# Autodesk Inventor assembly: Ensamblaje1
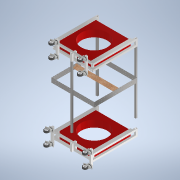
[picture p0: Inventor's stored thumbnail of the model, 180x180]
Saved by Autodesk Inventor 2020 (Build 240168000, 168)
## iProperties
Created: 2022-03-23
Part Number: Ensamblaje1
Document SubType Name: Assembly
Designer: aarco
Author: aarco
## Documents named in this file (8)
- C:\Users\aarco\Desktop\IDOM\Ensamblaje1.iam
- C:\Users\aarco\Desktop\IDOM\Latch.ipt
- C:\Users\aarco\Desktop\IDOM\SoporteBobina.ipt
- C:\Users\aarco\Desktop\IDOM\Madera.ipt
- C:\Users\aarco\Desktop\IDOM\Bobina.ipt
- C:\Users\aarco\Desktop\IDOM\Grid.ipt
- C:\Users\aarco\Desktop\IDOM\SoporteBobina_izq.ipt
- C:\Users\aarco\Desktop\IDOM\BPAB 1001 6150.ipt
## Components (18 placed, 7 different names)
1. Latch:1 — Rígido:1
2. SoporteBobina:1 — Coincidencia:1, Coincidencia:3, Coincidencia:4, Nivelación:1, Coincidencia:5, Coincidencia:7, Coincidencia:18, Nivelación:9, Nivelación:10, Coincidencia:24, Nivelación:13, Nivelación:14
3. Madera:1 — Rígido:1, Rígido:2, Coincidencia:13, Ángulo:1, Rígido:3, Rígido:4, Coincidencia:14, Coincidencia:15, Nivelación:8
4. Latch:2 — Rígido:2
5. Bobina:1 — Coincidencia:1, Coincidencia:3, Coincidencia:4
6. Grid:1 — Coincidencia:14, Coincidencia:15, Nivelación:8, Coincidencia:17, Coincidencia:18, Coincidencia:25
7. Bobina:2 — Coincidencia:20, Coincidencia:21, Coincidencia:22
8. Latch:3 — Rígido:3
9. Latch:4 — Rígido:4
10. SoporteBobina_izq:1 — Nivelación:9, Nivelación:10, Coincidencia:20, Coincidencia:21, Coincidencia:22, Coincidencia:23, Nivelación:11, Nivelación:12, Coincidencia:25
11. BPAB 1001 6150:1 — Coincidencia:23, Nivelación:11, Nivelación:12
12. BPAB 1001 6150:2
13. BPAB 1001 6150:3
14. BPAB 1001 6150:4
15. BPAB 1001 6150:6 — Coincidencia:24, Nivelación:13, Nivelación:14
16. BPAB 1001 6150:7
17. BPAB 1001 6150:8
18. BPAB 1001 6150:9
## Component patterns: (4 elements, first: BPAB 1001 6150:1), (4 elements, first: BPAB 1001 6150:6)
## Relationships (29: Mate 16, Flush 8, WeldJoint 4, Angle 1)
- Rígido:1 [WeldJoint]: Latch:1 ↔ Madera:1
- Rígido:2 [WeldJoint]: Madera:1 ↔ Latch:2
- Coincidencia:1 [Mate]: SoporteBobina:1 ↔ Bobina:1
- Coincidencia:3 [Mate]: SoporteBobina:1 ↔ Bobina:1
- Coincidencia:4 [Mate]: SoporteBobina:1 ↔ Bobina:1
- Nivelación:1 [Flush] (500 mm): SoporteBobina:1
- Coincidencia:5 [Mate]: SoporteBobina:1
- Coincidencia:7 [Mate]: SoporteBobina:1
- Coincidencia:13 [Mate]: Madera:1
- Ángulo:1 [Angle] (0 deg): Madera:1
- Rígido:3 [WeldJoint]: Madera:1 ↔ Latch:3
- Rígido:4 [WeldJoint]: Madera:1 ↔ Latch:4
- Coincidencia:14 [Mate]: Madera:1 ↔ Grid:1
- Coincidencia:15 [Mate] (400 mm): Madera:1 ↔ Grid:1
- Nivelación:8 [Flush]: Madera:1 ↔ Grid:1
- Coincidencia:17 [Mate]: Grid:1
- Coincidencia:18 [Mate] (800 mm): SoporteBobina:1 ↔ Grid:1
- Nivelación:9 [Flush]: SoporteBobina:1 ↔ SoporteBobina_izq:1
- Nivelación:10 [Flush]: SoporteBobina:1 ↔ SoporteBobina_izq:1
- Coincidencia:20 [Mate]: Bobina:2 ↔ SoporteBobina_izq:1
- Coincidencia:21 [Mate]: Bobina:2 ↔ SoporteBobina_izq:1
- Coincidencia:22 [Mate]: Bobina:2 ↔ SoporteBobina_izq:1
- Coincidencia:23 [Mate]: SoporteBobina_izq:1 ↔ BPAB 1001 6150:1
- Nivelación:11 [Flush] (-2.5 mm): SoporteBobina_izq:1 ↔ BPAB 1001 6150:1
- Nivelación:12 [Flush] (2.5 mm): SoporteBobina_izq:1 ↔ BPAB 1001 6150:1
- Coincidencia:24 [Mate]: SoporteBobina:1 ↔ BPAB 1001 6150:6
- Nivelación:13 [Flush] (2.5 mm): SoporteBobina:1 ↔ BPAB 1001 6150:6
- Nivelación:14 [Flush] (-2.5 mm): SoporteBobina:1 ↔ BPAB 1001 6150:6
- Coincidencia:25 [Mate]: Grid:1 ↔ SoporteBobina_izq:1
